# Autodesk Inventor assembly: Drive_Link_COG
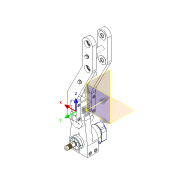
[picture p0: Inventor's stored thumbnail of the model, 180x180]
Saved by Autodesk Inventor 2022 (Build 260153000, 153)
## iProperties
Created: 2022-10-18
Part Number: Drive_Link_COG
Document SubType Name: Assembly
Designer: alexw
Mass: 1064.37 g
Surface Area: 1497.42 cm^2
Volume: 456.326 cm^3
Density: 2.33248 g/cm^3
Author: alexw
## Documents named in this file (5)
- C:\Users\alexw\Documents\Inventor\Projects\03_CurrentProjects\MasterThesis\PSM_V1_Rillenkugellager\COG\Drive_Link_COG.iam
- C:\Users\alexw\Documents\Inventor\Projects\03_CurrentProjects\MasterThesis\PSM_V1_Rillenkugellager\ParallelMechanismus_Driven_Assembly_v2.1_Rillenkugellager_Anlaufscheibe.iam
- C:\Users\alexw\Documents\Inventor\Projects\03_CurrentProjects\MasterThesis\PSM_V1_Rillenkugellager\MorotFixation_CounterWeightHolder_Assembly.iam
- C:\Users\alexw\Documents\Inventor\Projects\03_CurrentProjects\MasterThesis\PSM_V1_Rillenkugellager\Shaft_6mmx62mm.ipt
- C:\Users\alexw\Documents\Inventor\Projects\03_CurrentProjects\MasterThesis\PSM_V1_Rillenkugellager\ContentCenter\de-DE\ISO 4762(2)\ISO 4762 - M4 x 25ISO.ipt
## Components (5 placed, 4 different names)
1. ParallelMechanismus_Driven_Assembly_v2.1_Rillenkugellager_Anlaufscheibe:1 [sub-assembly] — Passend:3, Fluchtend:1, Passend:8, Fluchtend:2, Fluchtend:3, Passend:9
2. MorotFixation_CounterWeightHolder_Assembly:1 [sub-assembly] — Passend:4, Passend:5, Passend:6, Passend:7, Passend:9, Passend:10
3. Shaft_6mmx62mm:1 — Passend:3, Fluchtend:1
4. ISO 4762 M4 x 25:1 — Passend:4, Passend:5
5. ISO 4762 M4 x 25:2 — Passend:6, Passend:7
## Relationships (13: Mate 10, Flush 3)
- [Mate]: ParallelMechanismus_Driven_Assembly_v2.1_Rillenkugellager_Anlaufscheibe:1 ↔ MorotFixation_CounterWeightHolder_Assembly:1
- [Mate]: ParallelMechanismus_Driven_Assembly_v2.1_Rillenkugellager_Anlaufscheibe:1 ↔ MorotFixation_CounterWeightHolder_Assembly:1
- Passend:3 [Mate]: ParallelMechanismus_Driven_Assembly_v2.1_Rillenkugellager_Anlaufscheibe:1 ↔ Shaft_6mmx62mm:1
- Fluchtend:1 [Flush]: ParallelMechanismus_Driven_Assembly_v2.1_Rillenkugellager_Anlaufscheibe:1 ↔ Shaft_6mmx62mm:1
- Passend:4 [Mate]: MorotFixation_CounterWeightHolder_Assembly:1 ↔ ISO 4762 M4 x 25:1
- Passend:5 [Mate]: MorotFixation_CounterWeightHolder_Assembly:1 ↔ ISO 4762 M4 x 25:1
- Passend:6 [Mate]: MorotFixation_CounterWeightHolder_Assembly:1 ↔ ISO 4762 M4 x 25:2
- Passend:7 [Mate]: MorotFixation_CounterWeightHolder_Assembly:1 ↔ ISO 4762 M4 x 25:2
- Passend:8 [Mate]: ParallelMechanismus_Driven_Assembly_v2.1_Rillenkugellager_Anlaufscheibe:1
- Fluchtend:2 [Flush]: ParallelMechanismus_Driven_Assembly_v2.1_Rillenkugellager_Anlaufscheibe:1
- Fluchtend:3 [Flush]: ParallelMechanismus_Driven_Assembly_v2.1_Rillenkugellager_Anlaufscheibe:1
- Passend:9 [Mate]: ParallelMechanismus_Driven_Assembly_v2.1_Rillenkugellager_Anlaufscheibe:1 ↔ MorotFixation_CounterWeightHolder_Assembly:1
- Passend:10 [Mate]: MorotFixation_CounterWeightHolder_Assembly:1
